# Autodesk Inventor assembly: 00_RGB_Laser_converted
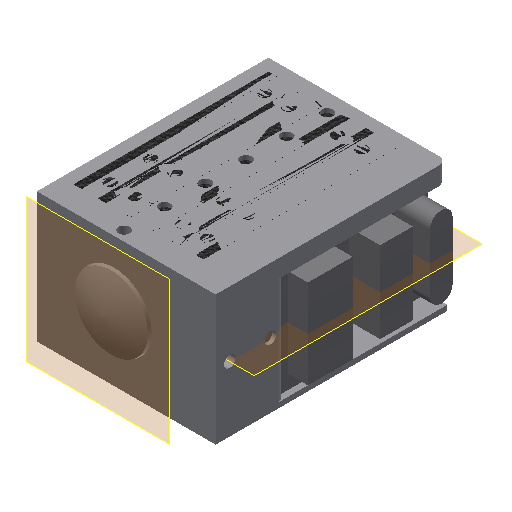
[picture p0: Inventor's stored thumbnail of the model, 512x512]
Saved by Autodesk Inventor 2022 (Build 260153000, 153)
## iProperties
Created: 2021-09-30
Part Number: 00_RGB_Laser_converted
Document SubType Name: Assembly
Designer: diederichbenedict
Author: diederichbenedict
## Documents named in this file (5)
- C:\Users\Muriel\Documents\GitHub\cellstorm\INVENTOR\00_RGB_Laser_converted.iam
- C:\Users\Muriel\Documents\GitHub\cellstorm\INVENTOR\00_RGB_Laser_Laserlands.ipt
- C:\Users\Muriel\Documents\GitHub\cellstorm\INVENTOR\00_LASER_640nm.ipt
- C:\Users\Muriel\Documents\GitHub\cellstorm\INVENTOR\00_lens_f25mm.ipt
- C:\Users\Muriel\Documents\GitHub\cellstorm\INVENTOR\00_RGB_Red_Laser_converter.ipt
## Components (4 placed, 4 different names)
1. 00_RGB_Laser_Laserlands:1 — Insert:2, Angle:1, Insert:3, Flush:1
2. 00_LASER_640nm:1 — Insert:2, Angle:1, Flush:2
3. 00_lens_f25mm:1 — Insert:3
4. 00_RGB_Red_Laser_converter:1 — Flush:1, Flush:2
## Relationships (5: Insert 2, Flush 2, Angle 1)
- Insert:2: 00_RGB_Laser_Laserlands:1 ↔ 00_LASER_640nm:1
- Angle:1 (180 deg): 00_RGB_Laser_Laserlands:1 ↔ 00_LASER_640nm:1
- Insert:3 (2 mm): 00_RGB_Laser_Laserlands:1 ↔ 00_lens_f25mm:1
- Flush:1: 00_RGB_Laser_Laserlands:1 ↔ 00_RGB_Red_Laser_converter:1
- Flush:2 (10 mm): 00_LASER_640nm:1 ↔ 00_RGB_Red_Laser_converter:1
